# Autodesk Inventor assembly: chain 3.48
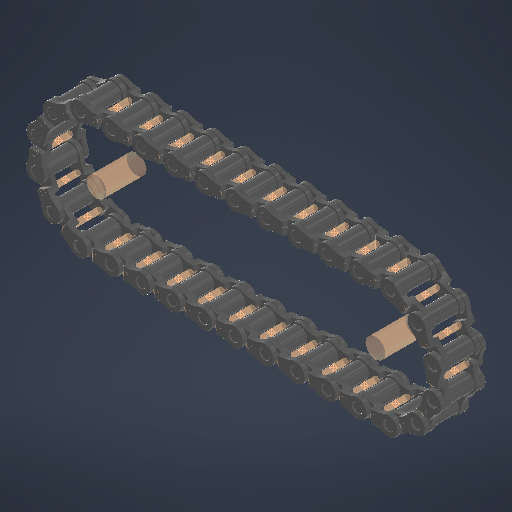
[picture p0: Inventor's stored thumbnail of the model, 512x512]
Saved by Autodesk Inventor 2025.2 (Build 292293000, 293)
## iProperties
Created: 2025-12-05
Part Number: chain 3.48
Document SubType Name: Assembly
Designer: cloudy
Author: cloudy
## Documents named in this file (3)
- C:\Users\cloudy\Documents\GitHub\aura-cad\15\chain 3.48.iam
- C:\Users\cloudy\Documents\GitHub\aura-cad\15\chain3.48path.ipt
- C:\Users\cloudy\Documents\GitHub\aura-cad\!lib\Motion\Chain 9P\High Strength Chain Link.ipt
## Components (31 placed, 2 different names)
1. chain3.48path:1 — Mate:2, Angle:1
2. High Strength Chain Link:1 — Mate:1, Mate:2, Angle:1
3. High Strength Chain Link:2
4. High Strength Chain Link:3
5. High Strength Chain Link:4
6. High Strength Chain Link:5
7. High Strength Chain Link:6
8. High Strength Chain Link:7
9. High Strength Chain Link:8
10. High Strength Chain Link:9
11. High Strength Chain Link:10
12. High Strength Chain Link:11
13. High Strength Chain Link:12
14. High Strength Chain Link:13
15. High Strength Chain Link:14
16. High Strength Chain Link:15
17. High Strength Chain Link:16
18. High Strength Chain Link:17
19. High Strength Chain Link:18
20. High Strength Chain Link:19
21. High Strength Chain Link:20
22. High Strength Chain Link:21
23. High Strength Chain Link:22
24. High Strength Chain Link:23
25. High Strength Chain Link:24
26. High Strength Chain Link:25
27. High Strength Chain Link:26
28. High Strength Chain Link:27
29. High Strength Chain Link:28
30. High Strength Chain Link:29
31. High Strength Chain Link:30
## Component patterns: (30 elements, first: High Strength Chain Link:1)
## Relationships (3: Mate 2, Angle 1)
- Mate:1: High Strength Chain Link:1
- Mate:2: chain3.48path:1 ↔ High Strength Chain Link:1
- Angle:1 (90 deg): chain3.48path:1 ↔ High Strength Chain Link:1
